# Autodesk Inventor assembly: box
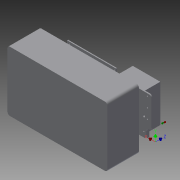
[picture p0: Inventor's stored thumbnail of the model, 180x180]
Saved by Autodesk Inventor 2015 (Build 190159000, 159)
## iProperties
Created: 2015-07-23
Part Number: box
Document SubType Name: Assembly
Designer: Simen
Author: Simen
## Documents named in this file (7)
- C:\Users\Simen\Documents\Inventor\lysreklemen\box.iam
- C:\Users\Simen\Documents\Inventor\lysreklemen\boks.ipt
- C:\Users\Simen\Documents\Inventor\lysreklemen\bakplate.ipt
- C:\Users\Simen\Documents\Inventor\lysreklemen\power_suply.ipt
- C:\Users\Simen\Documents\Inventor\lysreklemen\konektor kort.ipt
- C:\Users\Simen\Documents\Inventor\lysreklemen\contorller kort.ipt
- C:\Users\Simen\Documents\Inventor\lysreklemen\driver kort.ipt
## Components (6 placed, 6 different names)
1. boks:1
2. bakplate:1 — Mate:3, Mate:4, Flush:8, Flush:9, Flush:10, Flush:11
3. power_suply:1 — Mate:3, Flush:10, Flush:11
4. konektor kort:1 — Flush:3, Mate:2, Flush:4, Flush:5
5. contorller kort:1 — Flush:3, Mate:2, Flush:4, Flush:6, Flush:7, Flush:9
6. driver kort:1 — Flush:5, Flush:6, Flush:7, Mate:4, Flush:8
## Relationships (12: Flush 9, Mate 3)
- Flush:3: konektor kort:1 ↔ contorller kort:1
- Mate:2 (8 mm): konektor kort:1 ↔ contorller kort:1
- Flush:4: konektor kort:1 ↔ contorller kort:1
- Flush:5: konektor kort:1 ↔ driver kort:1
- Flush:6: contorller kort:1 ↔ driver kort:1
- Flush:7: contorller kort:1 ↔ driver kort:1
- Mate:3: bakplate:1 ↔ power_suply:1
- Mate:4 (10 mm): bakplate:1 ↔ driver kort:1
- Flush:8: bakplate:1 ↔ driver kort:1
- Flush:9: bakplate:1 ↔ contorller kort:1
- Flush:10: bakplate:1 ↔ power_suply:1
- Flush:11: bakplate:1 ↔ power_suply:1
